# Autodesk Inventor assembly: E005-Bielle
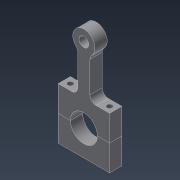
[picture p0: Inventor's stored thumbnail of the model, 180x180]
Saved by Autodesk Inventor 2021.3 (Build 253353000, 353)
## iProperties
Created: 2022-03-31
Part Number: E005-Bielle
Document SubType Name: Assembly
Designer: remi
Author: remi
## Documents named in this file (3)
- C:\Users\remi\OneDrive\Documents\Cours\05-HEVS\S2fb\mechanic\CCo\project\Compressor\E005-Bielle.iam
- C:\Users\remi\OneDrive\Documents\Cours\05-HEVS\S2fb\mechanic\CCo\project\Compressor\P012-Corps_bielle.ipt
- C:\Users\remi\OneDrive\Documents\Cours\05-HEVS\S2fb\mechanic\CCo\project\Compressor\P014-Chapeau_bielle.ipt
## Components (2 placed, 2 different names)
1. P012-Corps_bielle:1 — Mate:1, Mate:2, Mate:3
2. P014-Chapeau_bielle:1 — Mate:1, Mate:2, Mate:3
## Relationships (3: Mate 3)
- Mate:1: P012-Corps_bielle:1 ↔ P014-Chapeau_bielle:1
- Mate:2: P012-Corps_bielle:1 ↔ P014-Chapeau_bielle:1
- Mate:3: P012-Corps_bielle:1 ↔ P014-Chapeau_bielle:1
